# Autodesk Inventor assembly: linac_150mm_1500N-asm
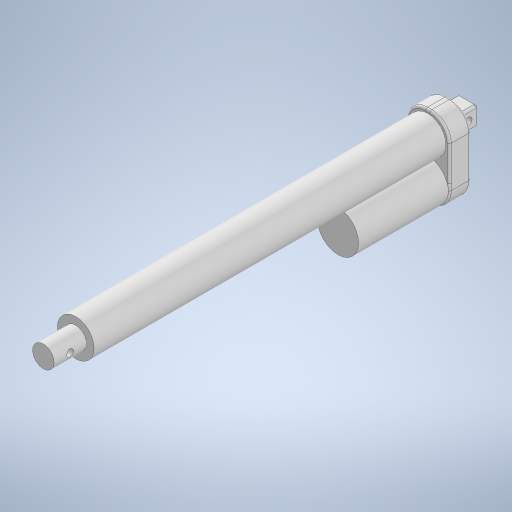
[picture p0: Inventor's stored thumbnail of the model, 512x512]
Saved by Autodesk Inventor 2024 (Build 280153000, 153)
## iProperties
Created: 2025-12-25
Part Number: linac_150mm_1500N-asm
Document SubType Name: Assembly
Designer: schar
Author: schar
## Documents named in this file (3)
- C:\Users\schar\Desktop\projectBlueprint\AMSTS\hardware\linac_150mm_1500N-asm.iam
- C:\Users\schar\Desktop\projectBlueprint\AMSTS\hardware\linac_150mm_1500N_outer.ipt
- C:\Users\schar\Desktop\projectBlueprint\AMSTS\hardware\linac_150mm_1500N_inner.ipt
## Components (2 placed, 2 different names)
1. linac_150mm_1500N_outer:2 — Cylindrical:1
2. linac_150mm_1500N_inner:1 — Cylindrical:1
## Relationships (1: CylindricalJoint 1)
- Cylindrical:1: linac_150mm_1500N_outer:2 ↔ linac_150mm_1500N_inner:1
